# Autodesk Inventor assembly: foot_parts
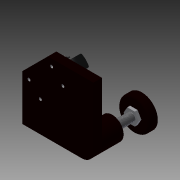
[picture p0: Inventor's stored thumbnail of the model, 180x180]
Saved by Autodesk Inventor 2015 (Build 190159000, 159)
## iProperties
Created: 2015-12-24
Part Number: foot_parts
Document SubType Name: Assembly
Designer: Ryo
Author: Ryo
## Documents named in this file (4)
- D:\Users\Ryo\Documents\Inventor\motoman_cad\SIA5_TABLE\INVENTOR2015\foot_parts.iam
- D:\Users\Ryo\Documents\Inventor\motoman_cad\SIA5_TABLE\INVENTOR2015\foot.ipt
- D:\Users\Ryo\Documents\Inventor\motoman_cad\SIA5_TABLE\parts\CHAMJ-E50-R.iam
- D:\Users\Ryo\Documents\Inventor\Content Center Files\R2015\ja-JP\JIS B 1176\JIS B 1176 - M6 x 10.ipt
## Components (6 placed, 3 different names)
1. foot:1 — メイト:1, メイト:2, メイト:3
2. CHAMJ-E50-R:1 [sub-assembly] — メイト:1, メイト:2, メイト:3, 挿入:1, 挿入:2, 挿入:3, 挿入:4
3. JIS B 1176 - メートル M6 x 10:1 — 挿入:1
4. JIS B 1176 - メートル M6 x 10:2 — 挿入:2
5. JIS B 1176 - メートル M6 x 10:3 — 挿入:3
6. JIS B 1176 - メートル M6 x 10:4 — 挿入:4
## Relationships (7: Insert 4, Mate 3)
- メイト:1 [Mate]: foot:1 ↔ CHAMJ-E50-R:1
- メイト:2 [Mate]: foot:1 ↔ CHAMJ-E50-R:1
- メイト:3 [Mate]: foot:1 ↔ CHAMJ-E50-R:1
- 挿入:1 [Insert]: CHAMJ-E50-R:1 ↔ JIS B 1176 - メートル M6 x 10:1
- 挿入:2 [Insert]: CHAMJ-E50-R:1 ↔ JIS B 1176 - メートル M6 x 10:2
- 挿入:3 [Insert]: CHAMJ-E50-R:1 ↔ JIS B 1176 - メートル M6 x 10:3
- 挿入:4 [Insert]: CHAMJ-E50-R:1 ↔ JIS B 1176 - メートル M6 x 10:4
